# Autodesk Inventor assembly: TPU Based Assembly
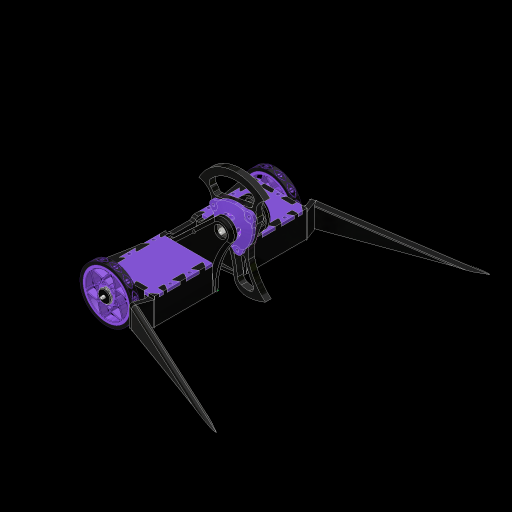
[picture p0: Inventor's stored thumbnail of the model, 512x512]
Saved by Autodesk Inventor 2023 (Build 270158000, 158)
## iProperties
Created: 2022-02-23
Part Number: TPU Based Assembly
Document SubType Name: Assembly
Designer: tandu
Mass: 457.507 g
Surface Area: 1504.43 cm^2
Volume: 256.612 cm^3
Density: 1.78288 g/cm^3
Author: tandu
## Documents named in this file (24)
- C:\Users\tandu\Documents\GrabCAD\Insomnia 2020\Versions\11 Wheel Guards and AR500 Blade\TPU Based Assembly 9.iam
- C:\Users\tandu\Documents\GrabCAD\Insomnia 2020\Versions\11 Wheel Guards and AR500 Blade\BatteryMockup.ipt
- C:\Users\tandu\Documents\GrabCAD\Insomnia 2020\Versions\11 Wheel Guards and AR500 Blade\CorrectSizeWheelsIThink.ipt
- C:\Users\tandu\Documents\GrabCAD\Insomnia 2020\Versions\11 Wheel Guards and AR500 Blade\EMax RS2205 v1.ipt
- C:\Users\tandu\Documents\GrabCAD\Insomnia 2020\Versions\11 Wheel Guards and AR500 Blade\FingerTech_Silver_Spark_223350.ipt
- C:\Users\tandu\Documents\GrabCAD\Insomnia 2020\Versions\11 Wheel Guards and AR500 Blade\TPU 22 Chassis.ipt
- C:\Users\tandu\Documents\GrabCAD\Insomnia 2020\Versions\11 Wheel Guards and AR500 Blade\UHMWMotorUpright.ipt
- C:\Users\tandu\Documents\GrabCAD\Insomnia 2020\Versions\11 Wheel Guards and AR500 Blade\UHMWBearingUpright.ipt
- C:\Users\tandu\Documents\GrabCAD\Insomnia 2020\Versions\11 Wheel Guards and AR500 Blade\OldBlade\Aluminimumanfmonfo Jank Weapon Fix.iam
- C:\Users\tandu\Documents\GrabCAD\Insomnia 2020\Versions\11 Wheel Guards and AR500 Blade\WedgeUHMWPiece.ipt
- C:\Users\tandu\Documents\GrabCAD\Insomnia 2020\Versions\11 Wheel Guards and AR500 Blade\57155K571_Flanged Ball Bearing.ipt
- C:\Users\tandu\Documents\GrabCAD\Insomnia 2020\Versions\11 Wheel Guards and AR500 Blade\2207 5 fixed motor.ipt
- C:\Users\tandu\Documents\GrabCAD\Insomnia 2020\Versions\11 Wheel Guards and AR500 Blade\WeaponSpacer.ipt
- C:\Users\tandu\Documents\GrabCAD\Insomnia 2020\Versions\11 Wheel Guards and AR500 Blade\WedgeUHMWPiece_MIR.ipt
- C:\Users\tandu\Documents\GrabCAD\Insomnia 2020\Versions\11 Wheel Guards and AR500 Blade\Derived Lid v8.ipt
- C:\Users\tandu\Documents\GrabCAD\Insomnia 2020\Versions\11 Wheel Guards and AR500 Blade\90417A126_Phillips Rounded Head Thread-Forming Screws.ipt
- E:\Users\tandu\Documents\GrabCAD\Insomnia 2020\Versions\9 Comically Large Weapon 9 28 22\FT Clamping Weapon\Viper-V-Spinner-Add-On.iam
- E:\Users\tandu\Documents\GrabCAD\Insomnia 2020\Versions\9 Comically Large Weapon 9 28 22\TPUWeapon\TPUWeaponAssembly.iam
- C:\Users\tandu\Documents\GrabCAD\Insomnia 2020\Versions\11 Wheel Guards and AR500 Blade\AR500 Weapon\AR500 Blade.ipt
- C:\Users\tandu\Documents\GrabCAD\Insomnia 2020\Versions\11 Wheel Guards and AR500 Blade\AR500 Weapon\PocketedSymmetrical\Pocketed Symetrical AR500 Blade.ipt
- C:\Users\tandu\Documents\GrabCAD\Insomnia 2020\Versions\11 Wheel Guards and AR500 Blade\NewWheels\banebots 3mm hub.iam
- C:\Users\tandu\Documents\GrabCAD\Insomnia 2020\Versions\11 Wheel Guards and AR500 Blade\NewWheels\NewWheelCore.ipt
- C:\Users\tandu\Documents\GrabCAD\Insomnia 2020\Versions\11 Wheel Guards and AR500 Blade\AR500 Weapon\TPUWeaponHubForAR500Blades.ipt
- C:\Users\tandu\Documents\GrabCAD\Insomnia 2020\Versions\11 Wheel Guards and AR500 Blade\AR500 Weapon\Fixed TPU Weapon Hub For AR500 Blades.ipt
## Components (29 placed, 23 different names)
1. BatteryMockup:1 — Mate:1, Mate:6, Mate:7
2. CorrectSizeWheelsIThink:1 — Insert:2
3. FingerTech_Silver_Spark_223350:1 — Insert:9, Mate:4
4. TPU 22 Chassis:1 — Mate:1, Insert:1, Insert:2, Insert:9, Mate:4, Insert:10, Mate:5, Insert:11, Insert:12, Insert:13, Insert:14, Insert:18, Insert:19, Insert:20, Insert:21, Mate:6, Mate:7, Insert:26, Insert:27, Insert:30, Insert:31, Insert:32, Insert:33, Insert:34, Insert:36
5. FingerTech_Silver_Spark_223350:2 — Insert:10, Mate:5
6. CorrectSizeWheelsIThink:2 — Insert:1, Tangent:1
7. UHMWMotorUpright:1 — Insert:11, Insert:12, Insert:15, Insert:16, Insert:23, Insert:24, Symmetry:1, Insert:28
8. UHMWBearingUpright:1 — Insert:13, Insert:14, Insert:22, Symmetry:1
9. EMax RS2205 v1:1 — Insert:15, Insert:16
10. Aluminimumanfmonfo Jank Weapon Fix:1 [sub-assembly] — Insert:25
11. WedgeUHMWPiece:1 — Insert:20, Insert:21
12. WedgeUHMWPiece:2 — Insert:18, Insert:19, Mate:8
13. 57155K571_Flanged Ball Bearing:1 — Insert:22
14. 2207 5 fixed motor:1 — Insert:23, Insert:24, Insert:25, Mate:11, Insert:29, Insert:35
15. WeaponSpacer:1
16. WedgePiece_MIR:1 — Insert:30, Insert:31
17. Derived Lid v8:1 — Insert:26, Insert:27
18. 90417A126_Phillips Rounded Head Thread-Forming Screws:1 — Insert:28
19. Viper-V-Spinner-Add-On:1 [sub-assembly] — Mate:11, Flush:1
20. TPUWeaponAssembly:1 [sub-assembly] — Insert:29
21. Derived Lid v8:2 — Insert:32, Insert:33
22. AR500 Blade:1 — Mate:21, Mate:22, Mate:23, Insert:37, Insert:38
23. Pocketed Symetrical AR500 Blade:1 — Mate:18, Mate:19, Mate:20
24. banebots 3mm hub:1 [sub-assembly] — Insert:34, Mate:12, Mate:13, Mate:14
25. NewWheelCore:1 — Mate:12, Mate:13, Mate:14
26. banebots 3mm hub:2 [sub-assembly] — Insert:36
27. NewWheelCore:2
28. TPUWeaponHubForAR500Blades:1 — Insert:35, Mate:18, Mate:19, Mate:20, Mate:21, Mate:22, Mate:23
29. Fixed TPU Weapon Hub For AR500 Blades:1 — Insert:37, Insert:38
## Relationships (54: Insert 31, Mate 20, Symmetry 1, Tangent 1, Flush 1)
- Mate:1: BatteryMockup:1 ↔ TPU 22 Chassis:1
- Insert:1: TPU 22 Chassis:1 ↔ CorrectSizeWheelsIThink:2
- Insert:2: CorrectSizeWheelsIThink:1 ↔ TPU 22 Chassis:1
- Insert:9: FingerTech_Silver_Spark_223350:1 ↔ TPU 22 Chassis:1
- Mate:4: FingerTech_Silver_Spark_223350:1 ↔ TPU 22 Chassis:1
- Insert:10: TPU 22 Chassis:1 ↔ FingerTech_Silver_Spark_223350:2
- Mate:5: TPU 22 Chassis:1 ↔ FingerTech_Silver_Spark_223350:2
- Insert:11: TPU 22 Chassis:1 ↔ UHMWMotorUpright:1
- Insert:12: TPU 22 Chassis:1 ↔ UHMWMotorUpright:1
- Insert:13: TPU 22 Chassis:1 ↔ UHMWBearingUpright:1
- Insert:14: TPU 22 Chassis:1 ↔ UHMWBearingUpright:1
- Insert:15: UHMWMotorUpright:1 ↔ EMax RS2205 v1:1
- Insert:16: UHMWMotorUpright:1 ↔ EMax RS2205 v1:1
- Insert:18: TPU 22 Chassis:1 ↔ WedgeUHMWPiece:2
- Insert:19: TPU 22 Chassis:1 ↔ WedgeUHMWPiece:2
- Insert:20: TPU 22 Chassis:1 ↔ WedgeUHMWPiece:1
- Insert:21: TPU 22 Chassis:1 ↔ WedgeUHMWPiece:1
- Insert:22: UHMWBearingUpright:1 ↔ 57155K571_Flanged Ball Bearing:1
- Insert:23: UHMWMotorUpright:1 ↔ 2207 5 fixed motor:1
- Insert:24: UHMWMotorUpright:1 ↔ 2207 5 fixed motor:1
- Insert:25: Aluminimumanfmonfo Jank Weapon Fix:1 ↔ 2207 5 fixed motor:1
- Mate:6: BatteryMockup:1 ↔ TPU 22 Chassis:1
- Mate:7: BatteryMockup:1 ↔ TPU 22 Chassis:1
- Symmetry:1: UHMWMotorUpright:1 ↔ UHMWBearingUpright:1
- Mate:8: WedgeUHMWPiece:2
- Mate:10
- Tangent:1: CorrectSizeWheelsIThink:2
- Insert:26: TPU 22 Chassis:1 ↔ Derived Lid v8:1
- Insert:27: TPU 22 Chassis:1 ↔ Derived Lid v8:1
- Insert:28: UHMWMotorUpright:1 ↔ 90417A126_Phillips Rounded Head Thread-Forming Screws:1
- Mate:11: 2207 5 fixed motor:1 ↔ Viper-V-Spinner-Add-On:1
- Flush:1: Viper-V-Spinner-Add-On:1
- Insert:29: 2207 5 fixed motor:1 ↔ TPUWeaponAssembly:1
- Insert:30: TPU 22 Chassis:1 ↔ WedgePiece_MIR:1
- Insert:31: TPU 22 Chassis:1 ↔ WedgePiece_MIR:1
- Insert:32: TPU 22 Chassis:1 ↔ Derived Lid v8:2
- Insert:33: TPU 22 Chassis:1 ↔ Derived Lid v8:2
- Insert:34: TPU 22 Chassis:1 ↔ banebots 3mm hub:1
- Mate:12: banebots 3mm hub:1 ↔ NewWheelCore:1
- Mate:13: banebots 3mm hub:1 ↔ NewWheelCore:1
- Mate:14: banebots 3mm hub:1 ↔ NewWheelCore:1
- [Mate]: banebots 3mm hub:2 ↔ NewWheelCore:2
- [Mate]: banebots 3mm hub:2 ↔ NewWheelCore:2
- [Mate]: banebots 3mm hub:2 ↔ NewWheelCore:2
- Insert:35: 2207 5 fixed motor:1 ↔ TPUWeaponHubForAR500Blades:1
- Mate:18: Pocketed Symetrical AR500 Blade:1 ↔ TPUWeaponHubForAR500Blades:1
- Mate:19: Pocketed Symetrical AR500 Blade:1 ↔ TPUWeaponHubForAR500Blades:1
- Insert:36: TPU 22 Chassis:1 ↔ banebots 3mm hub:2
- Mate:20: Pocketed Symetrical AR500 Blade:1 ↔ TPUWeaponHubForAR500Blades:1
- Mate:21: AR500 Blade:1 ↔ TPUWeaponHubForAR500Blades:1
- Mate:22: AR500 Blade:1 ↔ TPUWeaponHubForAR500Blades:1
- Mate:23: AR500 Blade:1 ↔ TPUWeaponHubForAR500Blades:1
- Insert:37: AR500 Blade:1 ↔ Fixed TPU Weapon Hub For AR500 Blades:1
- Insert:38: AR500 Blade:1 ↔ Fixed TPU Weapon Hub For AR500 Blades:1
## Named parameters: d69_d66 = 0 mm, d70_d67 = 0 mm, d71_d68 = 0 mm
